# Autodesk Inventor assembly: Wheel_Truing
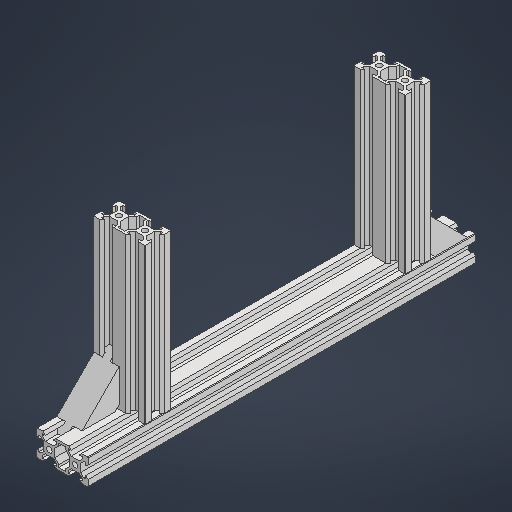
[picture p0: Inventor's stored thumbnail of the model, 512x512]
Saved by Autodesk Inventor 2026.1 (Build 301233020, 233B)
## iProperties
Created: 2025-12-18
Part Number: Wheel_Truing
Document SubType Name: Assembly
Designer: maciej
Author: maciej
## Documents named in this file (4)
- C:\Users\maciej\Desktop\studia\Labview\Wheel-Truing\Data\CAD\Wheel_Truing.iam
- C:\Users\maciej\Desktop\studia\Labview\Wheel-Truing\Data\CAD\2040vslot_short.ipt
- C:\Users\maciej\Desktop\studia\Labview\Wheel-Truing\Data\CAD\Kątownik.ipt
- C:\Users\maciej\Desktop\studia\Labview\Wheel-Truing\Data\CAD\2040vslot_long.ipt
## Components (5 placed, 3 different names)
1. 2040vslot_short:1 — Mate:6, Mate:7, Mate:10
2. Kątownik:1 — Mate:1, Mate:2, Mate:3, Mate:4
3. 2040vslot_long:1 — Mate:1, Mate:2, Mate:5, Mate:6, Mate:8, Mate:11
4. 2040vslot_short:2 — Mate:3, Mate:4, Mate:5
5. Kątownik:2 — Mate:7, Mate:8, Mate:10, Mate:11
## Relationships (10: Mate 10)
- Mate:1: Kątownik:1 ↔ 2040vslot_long:1
- Mate:2 (0.2 mm): Kątownik:1 ↔ 2040vslot_long:1
- Mate:3: Kątownik:1 ↔ 2040vslot_short:2
- Mate:4 (0.2 mm): Kątownik:1 ↔ 2040vslot_short:2
- Mate:5: 2040vslot_long:1 ↔ 2040vslot_short:2
- Mate:6: 2040vslot_short:1 ↔ 2040vslot_long:1
- Mate:7: 2040vslot_short:1 ↔ Kątownik:2
- Mate:8: 2040vslot_long:1 ↔ Kątownik:2
- Mate:10 (0.2 mm): 2040vslot_short:1 ↔ Kątownik:2
- Mate:11 (0.2 mm): 2040vslot_long:1 ↔ Kątownik:2
